# Autodesk Inventor assembly: Pully 34mmx8mm
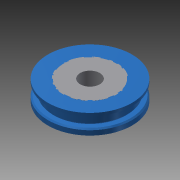
[picture p0: Inventor's stored thumbnail of the model, 180x180]
Saved by Autodesk Inventor 2013 (Build 170138000, 138)
## iProperties
Created: 2017-01-25
Part Number: Pully 34mmx8mm
Document SubType Name: Assembly
Designer: Herman de Vries
Author: Herman de Vries
## Documents named in this file (3)
- D:\Projects\Inventor\PaintBoid_2\Pully 34mmx8mm.iam
- D:\Projects\Inventor\PaintBoid_2\bearing 8mmx22mmx7mm.ipt
- D:\Projects\Inventor\PaintBoid_2\pully 22mmx34mmx8mm.ipt
## Components (2 placed, 2 different names)
1. bearing 8mmx22mmx7mm:1 — Insert:1
2. pully 22mmx34mmx8mm:1 — Insert:1
## Relationships (1: Insert 1)
- Insert:1: bearing 8mmx22mmx7mm:1 ↔ pully 22mmx34mmx8mm:1
